# Autodesk Inventor assembly: tip_3_n_base
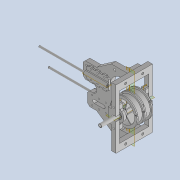
[picture p0: Inventor's stored thumbnail of the model, 180x180]
Saved by Autodesk Inventor 2020 (Build 240168000, 168)
## iProperties
Created: 2021-10-07
Part Number: tip_3_n_base
Document SubType Name: Assembly
Designer: Shuang Peng
Author: Shuang Peng
## Documents named in this file (8)
- D:\projects-3\torque fb tip\hardware\tip_3\tip_3_n_base.iam
- D:\projects-3\torque fb tip\hardware\tip_3\roller_4.ipt
- D:\projects-3\torque fb tip\hardware\tip_3\bearing_hh_1.ipt
- D:\projects-3\torque fb tip\hardware\tip_3\bearing_3_6_2.ipt
- D:\projects-3\torque fb tip\hardware\tip_3\pin3_40.ipt
- D:\projects-3\torque fb tip\hardware\tip_3\cpr_shell_1.ipt
- D:\projects-3\torque fb tip\hardware\tip_3\cpr_shell_2.ipt
- D:\projects-3\torque fb tip\hardware\tip_3\bl_tube_ass_2.iam
## Components (11 placed, 7 different names)
1. roller_4:1 — Insert:1, Insert:5
2. roller_4:2 — Insert:1, Insert:4
3. bearing_hh_1:1 — Insert:3, Flush:1, Flush:2, Flush:3, Insert:7
4. bearing_hh_1:2 — Insert:2, Flush:1
5. bearing_3_6_2:1 — Insert:2, Insert:5
6. bearing_3_6_2:2 — Insert:3, Insert:4, Insert:6
7. pin3_40:1 — Insert:6
8. cpr_shell_1:1 — Flush:2, Flush:3, Insert:7, Flush:4, Insert:8, Insert:9
9. cpr_shell_2:1 — Flush:4, Mate:1, Flush:5, Flush:6, Flush:8, Mate:2, Flush:9, Insert:8, Insert:9
10. bl_tube_ass_2:1 [sub-assembly] — Flush:8, Mate:2, Flush:9
11. bl_tube_ass_2:2 [sub-assembly] — Mate:1, Flush:5, Flush:6
## Relationships (19: Insert 9, Flush 8, Mate 2)
- Insert:1: roller_4:1 ↔ roller_4:2
- Insert:2: bearing_hh_1:2 ↔ bearing_3_6_2:1
- Insert:3: bearing_hh_1:1 ↔ bearing_3_6_2:2
- Insert:4: roller_4:2 ↔ bearing_3_6_2:2
- Insert:5: roller_4:1 ↔ bearing_3_6_2:1
- Flush:1: bearing_hh_1:1 ↔ bearing_hh_1:2
- Insert:6: bearing_3_6_2:2 ↔ pin3_40:1
- Flush:2: bearing_hh_1:1 ↔ cpr_shell_1:1
- Flush:3: bearing_hh_1:1 ↔ cpr_shell_1:1
- Insert:7: bearing_hh_1:1 ↔ cpr_shell_1:1
- Flush:4: cpr_shell_1:1 ↔ cpr_shell_2:1
- Mate:1: cpr_shell_2:1 ↔ bl_tube_ass_2:2
- Flush:5: cpr_shell_2:1 ↔ bl_tube_ass_2:2
- Flush:6 (10 mm): cpr_shell_2:1 ↔ bl_tube_ass_2:2
- Flush:8: cpr_shell_2:1 ↔ bl_tube_ass_2:1
- Mate:2: cpr_shell_2:1 ↔ bl_tube_ass_2:1
- Flush:9 (10 mm): cpr_shell_2:1 ↔ bl_tube_ass_2:1
- Insert:8: cpr_shell_1:1 ↔ cpr_shell_2:1
- Insert:9: cpr_shell_1:1 ↔ cpr_shell_2:1
